# Autodesk Inventor assembly: AxisY
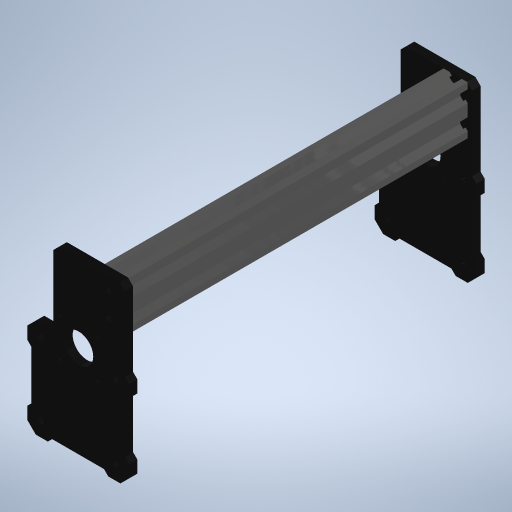
[picture p0: Inventor's stored thumbnail of the model, 512x512]
Saved by Autodesk Inventor 2024.3 (Build 283343000, 343)
## iProperties
Created: 2024-08-27
Part Number: AxisY
Document SubType Name: Assembly
Designer: Admin
Author: Admin
## Documents named in this file (3)
- C:\Users\migue\Documents\GitHub\RobotCartesiano\DiseñoBrazo\Assemblies\AxisY.iam
- C:\Users\migue\Documents\GitHub\RobotCartesiano\DiseñoBrazo\Axis\AxisY\AP-Y.ipt
- C:\Users\migue\Documents\GitHub\RobotCartesiano\DiseñoBrazo\AcrylicPieces\AxisY-Carrier.ipt
## Components (3 placed, 2 different names)
1. AP-Y:1 — Mate:1, Mate:2, Mate:3, Mate:4, Mate:5, Mate:6
2. AxisY-Carrier:1 — Mate:1, Mate:2, Mate:3
3. AxisY-Carrier:2 — Mate:4, Mate:5, Mate:6
## Relationships (6: Mate 6)
- Mate:1: AP-Y:1 ↔ AxisY-Carrier:1
- Mate:2: AP-Y:1 ↔ AxisY-Carrier:1
- Mate:3: AP-Y:1 ↔ AxisY-Carrier:1
- Mate:4: AP-Y:1 ↔ AxisY-Carrier:2
- Mate:5: AP-Y:1 ↔ AxisY-Carrier:2
- Mate:6: AP-Y:1 ↔ AxisY-Carrier:2
